# Autodesk Inventor assembly: PCB_board_assembly
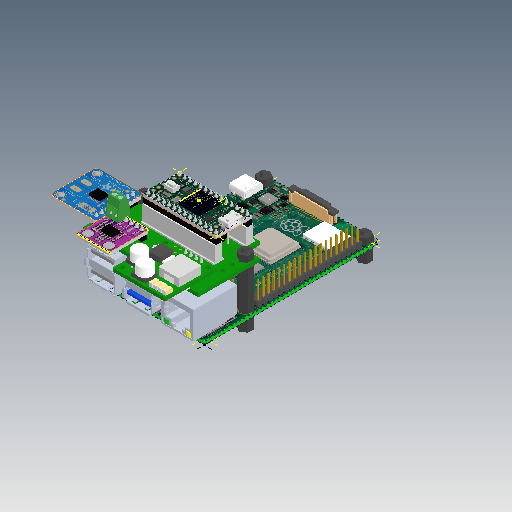
[picture p0: Inventor's stored thumbnail of the model, 512x512]
Saved by Autodesk Inventor 2020 (Build 240168000, 168)
## iProperties
Created: 2020-09-27
Part Number: PCB_board_assembly
Document SubType Name: Assembly
Designer: DELL
Mass: 33.6435 g
Surface Area: 486.264 cm^2
Volume: 33.6435 cm^3
Density: 1 g/cm^3
Author: DELL
## Documents named in this file (12)
- F:\SoftRobot\Model\FlexipodHardware-master\mechanical_model\PCB\PCB_board_assembly.iam
- F:\SoftRobot\Model\FlexipodHardware-master\mechanical_model\PCB\PCB_board\PCB.iam
- F:\SoftRobot\Model\FlexipodHardware-master\mechanical_model\PCB\teensy_4.0\teensy_4.0.iam
- F:\SoftRobot\Model\FlexipodHardware-master\mechanical_model\PCB\5V_5.5A_Voltage_Regulator_D36V50F5\voltage_regulator_with_pins.iam
- F:\SoftRobot\Model\FlexipodHardware-master\mechanical_model\PCB\Adafruit_INA260\INA260_with_pins.iam
- F:\SoftRobot\Model\FlexipodHardware-master\mechanical_model\PCB\CAN_transceiver\CAN_transceiver_with_pins.iam
- F:\SoftRobot\Model\FlexipodHardware-master\mechanical_model\PCB\capacitor.ipt
- F:\SoftRobot\Model\FlexipodHardware-master\mechanical_model\PCB\pins.ipt
- F:\SoftRobot\Model\FlexipodHardware-master\mechanical_model\PCB\raspberry_pi_4_b\raspberry_pi_4_model_B.iam
- F:\SoftRobot\Model\FlexipodHardware-master\mechanical_model\PCB\PCB_support\20mm_support.ipt
- F:\SoftRobot\Model\FlexipodHardware-master\mechanical_model\PCB\PCB_support\6mm_support.ipt
- F:\SoftRobot\Model\FlexipodHardware-master\mechanical_model\PCB\PCB_support\nut_support.ipt
## Components (19 placed, 11 different names)
1. PCB:1 [sub-assembly] — Mate:2, Flush:1, Mate:3, Mate:4, Mate:5, Mate:6, Mate:7, Mate:8, Mate:9, Mate:10, Mate:11, Mate:12, Mate:13, Mate:14, Tangent:1, Mate:15, Mate:16, Mate:17, Mate:18, Mate:19, Mate:20, Mate:23, Mate:24, Mate:26, Angle:2, Mate:40, Mate:43
2. teensy_4.0:1 [sub-assembly] — Mate:2, Flush:1, Mate:3
3. voltage_regulator_with_pins:1 [sub-assembly] — Mate:4, Mate:5, Mate:6
4. INA260_with_pins:1 [sub-assembly] — Mate:7, Mate:8, Mate:9
5. CAN_transceiver_with_pins:1 [sub-assembly] — Mate:10, Mate:11, Mate:12
6. capacitor:1 — Mate:13, Mate:14, Tangent:1
7. pins:1 — Mate:16, Mate:17, Flush:2
8. pins:2 — Mate:15, Mate:18, Flush:2
9. raspberry_pi_4_model_B:1 [sub-assembly] — Mate:19, Mate:20, Mate:21, Mate:22, Flush:3, Mate:25, Angle:1, Mate:27, Mate:28, Mate:29, Mate:30, Mate:31, Mate:32, Mate:33, Angle:5, Angle:6, Mate:34, Mate:35, Mate:37, Mate:39
10. 20mm_support:1 — Mate:23, Mate:24, Mate:25, Angle:1, Angle:3, Mate:42, Angle:10
11. 20mm_support:2 — Mate:26, Mate:27, Angle:2, Angle:4, Mate:41, Angle:9
12. 6mm_support:1 — Mate:28, Mate:30, Angle:3
13. 6mm_support:2 — Mate:29, Mate:31, Angle:4
14. 6mm_support:3 — Mate:32, Mate:33, Angle:5, Mate:36, Angle:7
15. 6mm_support:4 — Angle:6, Mate:34, Mate:35, Mate:38, Angle:8
16. nut_support:1 — Mate:36, Mate:37, Angle:7
17. nut_support:2 — Mate:38, Mate:39, Angle:8
18. nut_support:3 — Mate:42, Mate:43, Angle:10
19. nut_support:4 — Mate:40, Mate:41, Angle:9
## Relationships (56: Mate 42, Angle 10, Flush 3, Tangent 1)
- Mate:2: PCB:1 ↔ teensy_4.0:1
- Flush:1: PCB:1 ↔ teensy_4.0:1
- Mate:3: PCB:1 ↔ teensy_4.0:1
- Mate:4: PCB:1 ↔ voltage_regulator_with_pins:1
- Mate:5: PCB:1 ↔ voltage_regulator_with_pins:1
- Mate:6: PCB:1 ↔ voltage_regulator_with_pins:1
- Mate:7: PCB:1 ↔ INA260_with_pins:1
- Mate:8: PCB:1 ↔ INA260_with_pins:1
- Mate:9: PCB:1 ↔ INA260_with_pins:1
- Mate:10: PCB:1 ↔ CAN_transceiver_with_pins:1
- Mate:11: PCB:1 ↔ CAN_transceiver_with_pins:1
- Mate:12: PCB:1 ↔ CAN_transceiver_with_pins:1
- Mate:13: PCB:1 ↔ capacitor:1
- Mate:14: PCB:1 ↔ capacitor:1
- Tangent:1: PCB:1 ↔ capacitor:1
- Mate:15: PCB:1 ↔ pins:2
- Mate:16: PCB:1 ↔ pins:1
- Mate:17: PCB:1 ↔ pins:1
- Mate:18: PCB:1 ↔ pins:2
- Flush:2: pins:1 ↔ pins:2
- Mate:19: PCB:1 ↔ raspberry_pi_4_model_B:1
- Mate:20: PCB:1 ↔ raspberry_pi_4_model_B:1
- Mate:21: raspberry_pi_4_model_B:1
- Mate:22: raspberry_pi_4_model_B:1
- Flush:3: raspberry_pi_4_model_B:1
- Mate:23: PCB:1 ↔ 20mm_support:1
- Mate:24: PCB:1 ↔ 20mm_support:1
- Mate:25: raspberry_pi_4_model_B:1 ↔ 20mm_support:1
- Angle:1 (0 deg): raspberry_pi_4_model_B:1 ↔ 20mm_support:1
- Mate:26: PCB:1 ↔ 20mm_support:2
- Mate:27: raspberry_pi_4_model_B:1 ↔ 20mm_support:2
- Angle:2 (0 deg): PCB:1 ↔ 20mm_support:2
- Mate:28: raspberry_pi_4_model_B:1 ↔ 6mm_support:1
- Mate:29: raspberry_pi_4_model_B:1 ↔ 6mm_support:2
- Mate:30: raspberry_pi_4_model_B:1 ↔ 6mm_support:1
- Angle:3 (0 deg): 20mm_support:1 ↔ 6mm_support:1
- Mate:31: raspberry_pi_4_model_B:1 ↔ 6mm_support:2
- Angle:4 (0 deg): 20mm_support:2 ↔ 6mm_support:2
- Mate:32: raspberry_pi_4_model_B:1 ↔ 6mm_support:3
- Mate:33: raspberry_pi_4_model_B:1 ↔ 6mm_support:3
- Angle:5 (0 deg): raspberry_pi_4_model_B:1 ↔ 6mm_support:3
- Angle:6 (0 deg): raspberry_pi_4_model_B:1 ↔ 6mm_support:4
- Mate:34: raspberry_pi_4_model_B:1 ↔ 6mm_support:4
- Mate:35: raspberry_pi_4_model_B:1 ↔ 6mm_support:4
- Mate:36: 6mm_support:3 ↔ nut_support:1
- Mate:37: raspberry_pi_4_model_B:1 ↔ nut_support:1
- Angle:7 (0 deg): 6mm_support:3 ↔ nut_support:1
- Mate:38: 6mm_support:4 ↔ nut_support:2
- Mate:39: raspberry_pi_4_model_B:1 ↔ nut_support:2
- Angle:8 (0 deg): 6mm_support:4 ↔ nut_support:2
- Mate:40: PCB:1 ↔ nut_support:4
- Mate:41: 20mm_support:2 ↔ nut_support:4
- Angle:9 (0 deg): 20mm_support:2 ↔ nut_support:4
- Mate:42: 20mm_support:1 ↔ nut_support:3
- Mate:43: PCB:1 ↔ nut_support:3
- Angle:10 (0 deg): 20mm_support:1 ↔ nut_support:3
